# Autodesk Inventor assembly: Dowel Joint
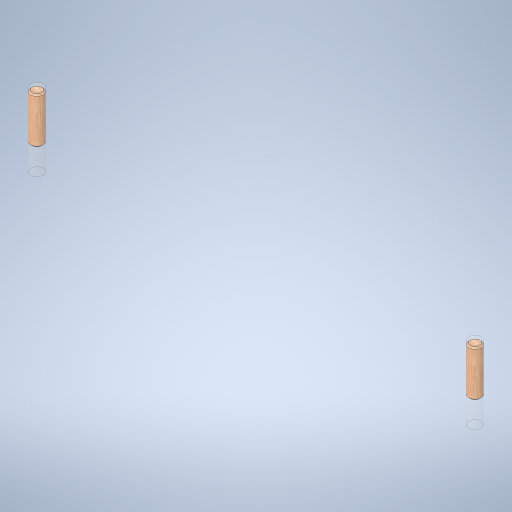
[picture p0: Inventor's stored thumbnail of the model, 512x512]
Saved by Autodesk Inventor 2024 (Build 280153000, 153)
## iProperties
RuleStatus: InUse
Created: 2023-02-13
Part Number: Dowel Joint
Document SubType Name: Assembly
Designer: sauliusd
Author: sauliusd
## Documents named in this file (3)
- C:\W4INV 2024 Design\SMART HARDWARE\Dowel Joint\Dowel Joint.iam
- C:\W4INV 2024 Design\SMART HARDWARE\Dowel Joint\Parts\Dowel Joint.ipt
- C:\W4INV 2024 Design\PROJECTS\MODEL STATE LIBRARY COMPONENTS\Dowel\MS Dowel.ipt
## Components (3 placed, 3 different names)
1. @Skeleton — Flush:1, Flush:2, Flush:3, Insert:1
2. Wood Dowel — Insert:1
3. MS Dowel:2
## Component patterns: (2 elements, first: Wood Dowel)
## Relationships (4: Flush 3, Insert 1)
- Flush:1: @Skeleton
- Flush:2: @Skeleton
- Flush:3: @Skeleton
- Insert:1: @Skeleton ↔ Wood Dowel
## Named parameters: ContactPatchWidth = 400 mm, ContactPatchHeight = 18 mm, NesteledBoardThickness = 18 mm, Gap = 0 mm, ConnectionAngle = 90 deg, MaxAllowedDistance = 500 mm, ShiftFromSide1 = 50 mm, ShiftFromSide2 = 50 mm, MinAllowedDistance = 20 mm, DowelD = 8 mm, DowelL = 30 mm, PillarBoardThickness = 18 mm, DrillTipOffset = 3 mm
